# Autodesk Inventor assembly: SD_BaseStation_Enclosure
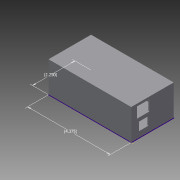
[picture p0: Inventor's stored thumbnail of the model, 180x180]
Saved by Autodesk Inventor 2015 (Build 190159000, 159)
## iProperties
Created: 2014-04-30
Part Number: SD_BaseStation_Enclosure
Document SubType Name: Assembly
Designer: xbmc
Author: xbmc
## Documents named in this file (3)
- C:\Users\xbmc\Desktop\SD_BaseStation_Enclosure.iam
- C:\Users\xbmc\Desktop\SD_BaseStation_Box.ipt
- C:\Users\xbmc\Desktop\SD_BaseStation_Lid.ipt
## Components (2 placed, 2 different names)
1. SD_BaseStation_Box:1 — Mate:1, Flush:1, Flush:2
2. SD_BaseStation_Lid:1 — Mate:1, Flush:1, Flush:2
## Relationships (3: Flush 2, Mate 1)
- Mate:1: SD_BaseStation_Box:1 ↔ SD_BaseStation_Lid:1
- Flush:1: SD_BaseStation_Box:1 ↔ SD_BaseStation_Lid:1
- Flush:2: SD_BaseStation_Box:1 ↔ SD_BaseStation_Lid:1
